# Autodesk Inventor assembly: full guns 3
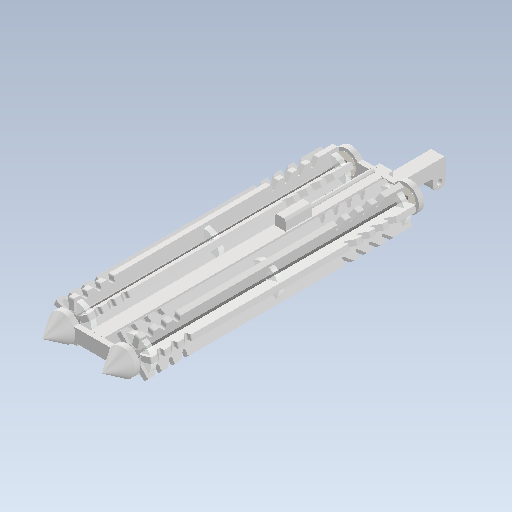
[picture p0: Inventor's stored thumbnail of the model, 512x512]
Saved by Autodesk Inventor 2020.1 (Build 241239000, 239)
## iProperties
Created: 2022-03-22
Part Number: full guns 3
Document SubType Name: Assembly
Designer: User
Author: User
## Documents named in this file (7)
- D:\GitHub\TANK\3D-turret\full guns 4.iam
- D:\GitHub\TANK\3D-turret\gun.iam
- D:\GitHub\TANK\3D-turret\подшипник.ipt
- D:\GitHub\TANK\3D-turret\соединение пушек перед.ipt
- D:\GitHub\TANK\3D-turret\соединение пушек.ipt
- D:\GitHub\TANK\3D-turret\центр пушки.ipt
- D:\GitHub\TANK\3D-turret\держак середины пушки ДЛИННАЯ ОЧЕНЬ.ipt
## Components (10 placed, 6 different names)
1. соединение пушек перед:2 — Жесткий:6, Жесткий:7, Жесткий:10
2. подшипник:6 — Жесткий:6, Вставка:2
3. gun:4 [sub-assembly] — Вставка:1
4. подшипник:8 — Жесткий:7, Вставка:1
5. gun:5 [sub-assembly] — Вставка:2
6. соединение пушек:1 — Жесткий:8, Жесткий:9, Жесткий:11, Жесткий:12
7. подшипник:9 — Жесткий:9
8. подшипник:10 — Жесткий:8
9. центр пушки:1 — Жесткий:10, Жесткий:11
10. держак середины пушки ДЛИННАЯ ОЧЕНЬ:1 — Жесткий:12
## Relationships (9: WeldJoint 7, Insert 2)
- Жесткий:6 [WeldJoint]: соединение пушек перед:2 ↔ подшипник:6
- Жесткий:7 [WeldJoint]: соединение пушек перед:2 ↔ подшипник:8
- Вставка:1 [Insert]: gun:4 ↔ подшипник:8
- Вставка:2 [Insert]: подшипник:6 ↔ gun:5
- Жесткий:8 [WeldJoint]: соединение пушек:1 ↔ подшипник:10
- Жесткий:9 [WeldJoint]: соединение пушек:1 ↔ подшипник:9
- Жесткий:10 [WeldJoint]: соединение пушек перед:2 ↔ центр пушки:1
- Жесткий:11 [WeldJoint]: соединение пушек:1 ↔ центр пушки:1
- Жесткий:12 [WeldJoint]: соединение пушек:1 ↔ держак середины пушки ДЛИННАЯ ОЧЕНЬ:1
